# Autodesk Inventor assembly: Snap_Switch_Assembly
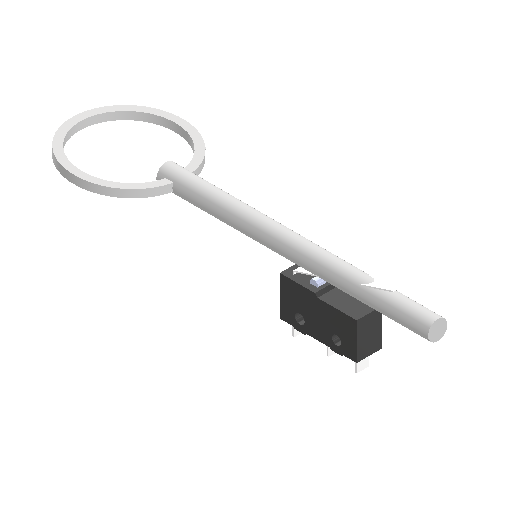
[picture p0: Inventor's stored thumbnail of the model, 512x512]
Saved by Autodesk Inventor 2026.2 (Build 302298010, 298A)
## iProperties
Created: 2026-02-23
Part Number: Snap_Switch_Assembly
Document SubType Name: Assembly
Designer: vckot
Author: vckot
## Documents named in this file (4)
- C:\Users\jocel\OneDrive\Desktop\1 - IBEHS 5P06 CAPSTONE\capstone\CAD_files\Version_6\Snap_Switch_Assembly.iam
- C:\Users\jocel\OneDrive\Desktop\1 - IBEHS 5P06 CAPSTONE\capstone\CAD_files\Version_6\SS-5FL111-3T.ipt
- C:\Users\jocel\OneDrive\Desktop\1 - IBEHS 5P06 CAPSTONE\capstone\CAD_files\Version_6\SS-5FL111-3T_Housing_01.ipt
- C:\Users\jocel\OneDrive\Desktop\1 - IBEHS 5P06 CAPSTONE\capstone\CAD_files\Version_6\SS-5FL111-3T_Housing_02.ipt
## Components (3 placed, 3 different names)
1. SS-5FL111-3T:1 — Mate:1, Mate:2, Flush:1
2. SS-5FL111-3T_Housing_01:1 — Mate:1, Mate:2, Flush:1, Mate:3, Mate:4
3. SS-5FL111-3T_Housing_02:1 — Mate:3, Mate:4
## Relationships (5: Mate 4, Flush 1)
- Mate:1: SS-5FL111-3T:1 ↔ SS-5FL111-3T_Housing_01:1
- Mate:2: SS-5FL111-3T:1 ↔ SS-5FL111-3T_Housing_01:1
- Flush:1: SS-5FL111-3T:1 ↔ SS-5FL111-3T_Housing_01:1
- Mate:3: SS-5FL111-3T_Housing_01:1 ↔ SS-5FL111-3T_Housing_02:1
- Mate:4 (5 mm): SS-5FL111-3T_Housing_01:1 ↔ SS-5FL111-3T_Housing_02:1
